# Autodesk Inventor assembly: CAM14
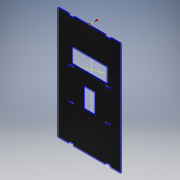
[picture p0: Inventor's stored thumbnail of the model, 180x180]
Saved by Autodesk Inventor 2017 (Build 210142000, 142)
## iProperties
Created: 2019-06-08
Part Number: CAM14
Document SubType Name: Assembly
Designer: Dell
Author: Dell
## Documents named in this file (2)
- C:\Users\Dell\Documents\GitHub\tr2\Body 2.0\CAM14.iam
- C:\Users\Dell\Documents\GitHub\tr2\Body 2.0\BA11.ipt
## Components (1 placed, 1 different names)
1. BA11:1 — Mate:1, Flush:1
## Relationships (2: Mate 1, Flush 1)
- Mate:1: BA11:1
- Flush:1: BA11:1
